# Autodesk Inventor assembly: Rama_siedziska
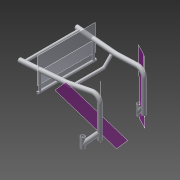
[picture p0: Inventor's stored thumbnail of the model, 180x180]
Saved by Autodesk Inventor 2015 (Build 190159000, 159)
## iProperties
Created: 2015-11-20
Part Number: Rama_siedziska
Document SubType Name: Konstrukcja spawana
Designer: graaapsik
Weld Material: Aluminium AW-7020
Author: graaapsik
## Documents named in this file (9)
- C:\Users\EriveltonDell\Documents\Centro Universitário da FEI\Wheelchair\CADEIRA DE RODAS - DESENHO\Model\Rama_siedziska.iam
- C:\Users\EriveltonDell\Documents\Centro Universitário da FEI\Wheelchair\CADEIRA DE RODAS - DESENHO\Model\Rura_podłużna_ergosiedziska_prawa.ipt
- C:\Users\EriveltonDell\Documents\Centro Universitário da FEI\Wheelchair\CADEIRA DE RODAS - DESENHO\Model\Rura_poprzeczna_ergosiedziska.ipt
- C:\Users\EriveltonDell\Documents\Centro Universitário da FEI\Wheelchair\CADEIRA DE RODAS - DESENHO\Model\Rura_poprzeczna_wygieta.ipt
- C:\Users\EriveltonDell\Documents\Centro Universitário da FEI\Wheelchair\CADEIRA DE RODAS - DESENHO\Model\Rura_podłużna_ergosiedziska_lewa.ipt
- C:\Users\EriveltonDell\Documents\Centro Universitário da FEI\Wheelchair\CADEIRA DE RODAS - DESENHO\Model\Rura_pionowa_kolka_przedniego.ipt
- C:\Users\EriveltonDell\Documents\Centro Universitário da FEI\Wheelchair\CADEIRA DE RODAS - DESENHO\Model\Rura_skosna_kolka_przedniego.ipt
- C:\Users\EriveltonDell\Documents\Centro Universitário da FEI\Wheelchair\CADEIRA DE RODAS - DESENHO\Model\Rura_pionowa_do_kol_tylnych.ipt
- C:\Users\EriveltonDell\Documents\Centro Universitário da FEI\Wheelchair\CADEIRA DE RODAS - DESENHO\Model\Belka.ipt
## Components (11 placed, 8 different names)
1. Rura_poprzeczna_ergosiedziska:1 — Równoległy:2, Równoległy:10, Zestawiający:1, Zestawiający:2, Zestawiający:3, Równoległy:11, Styczny:1, Zestawiający:4, Zestawiający:5, Zestawiający:7, Zestawiający:8, Zestawiający:29, Kąt:1
2. Rura_poprzeczna_wygieta:1 — Równoległy:10, Równoległy:12, Równoległy:13
3. Rura_podłużna_ergosiedziska_prawa:1 — Równoległy:2, Zestawiający:1, Zestawiający:2, Równoległy:13, Zestawiający:18, Zestawiający:22, Równoległy:14, Zestawiający:24, Zestawiający:25
4. Rura_podłużna_ergosiedziska_lewa:1 — Zestawiający:3, Równoległy:11, Styczny:1, Równoległy:12, Zestawiający:10, Zestawiający:16, Zestawiający:26, Zestawiający:27, Zestawiający:28, Równoległy:15
5. Rura_pionowa_kolka_przedniego:1 — Zestawiający:4, Zestawiający:5, Równoległy:16, Zestawiający:17, Zestawiający:23, Zestawiający:9
6. Rura_skosna_kolka_przedniego:1 — Zestawiający:21, Zestawiający:22, Zestawiający:23
7. Rura_pionowa_kolka_przedniego:2 — Zestawiający:7, Zestawiający:8, Zestawiający:9, Zestawiający:11, Zestawiający:15
8. Rura_skosna_kolka_przedniego:2 — Zestawiający:14, Zestawiający:15, Zestawiający:16
9. Rura_pionowa_do_kol_tylnych:1 — Równoległy:14, Zestawiający:24, Zestawiający:25, Symetria:1, Zestawiający:33
10. Rura_pionowa_do_kol_tylnych:2 — Zestawiający:26, Zestawiający:27, Zestawiający:28, Równoległy:15, Symetria:1, Zestawiający:32
11. Belka:1 — Zestawiający:29, Zestawiający:31, Równoległy:16
## Relationships (44: Mate 33, Flush 8, Tangent 1, Angle 1, Symmetry 1)
- Równoległy:2 [Flush]: Rura_poprzeczna_ergosiedziska:1 ↔ Rura_podłużna_ergosiedziska_prawa:1
- Równoległy:10 [Flush] (270 mm): Rura_poprzeczna_ergosiedziska:1 ↔ Rura_poprzeczna_wygieta:1
- Zestawiający:1 [Mate] (-30 mm): Rura_poprzeczna_ergosiedziska:1 ↔ Rura_podłużna_ergosiedziska_prawa:1
- Zestawiający:2 [Mate] (16 mm): Rura_poprzeczna_ergosiedziska:1 ↔ Rura_podłużna_ergosiedziska_prawa:1
- Zestawiający:3 [Mate] (-30 mm): Rura_poprzeczna_ergosiedziska:1 ↔ Rura_podłużna_ergosiedziska_lewa:1
- Równoległy:11 [Flush]: Rura_poprzeczna_ergosiedziska:1 ↔ Rura_podłużna_ergosiedziska_lewa:1
- Styczny:1 [Tangent]: Rura_poprzeczna_ergosiedziska:1 ↔ Rura_podłużna_ergosiedziska_lewa:1
- Równoległy:12 [Flush] (16 mm): Rura_poprzeczna_wygieta:1 ↔ Rura_podłużna_ergosiedziska_lewa:1
- Równoległy:13 [Flush] (16 mm): Rura_poprzeczna_wygieta:1 ↔ Rura_podłużna_ergosiedziska_prawa:1
- Zestawiający:4 [Mate] (450 mm): Rura_poprzeczna_ergosiedziska:1 ↔ Rura_pionowa_kolka_przedniego:1
- Zestawiający:5 [Mate] (-16 mm): Rura_poprzeczna_ergosiedziska:1 ↔ Rura_pionowa_kolka_przedniego:1
- Równoległy:16 [Flush] (-120 mm): Rura_pionowa_kolka_przedniego:1 ↔ Belka:1
- Zestawiający:7 [Mate] (416 mm): Rura_poprzeczna_ergosiedziska:1 ↔ Rura_pionowa_kolka_przedniego:2
- Zestawiający:8 [Mate] (450 mm): Rura_poprzeczna_ergosiedziska:1 ↔ Rura_pionowa_kolka_przedniego:2
- Zestawiający:9 [Mate]: Rura_pionowa_kolka_przedniego:1 ↔ Rura_pionowa_kolka_przedniego:2
- Zestawiający:10 [Mate]: Rura_podłużna_ergosiedziska_lewa:1
- Zestawiający:11 [Mate]: Rura_pionowa_kolka_przedniego:2
- Zestawiający:12 [Mate]
- Zestawiający:13 [Mate]
- Zestawiający:14 [Mate]: Rura_skosna_kolka_przedniego:2
- Zestawiający:15 [Mate] (16 mm): Rura_pionowa_kolka_przedniego:2 ↔ Rura_skosna_kolka_przedniego:2
- Zestawiający:16 [Mate] (16 mm): Rura_podłużna_ergosiedziska_lewa:1 ↔ Rura_skosna_kolka_przedniego:2
- Zestawiający:17 [Mate]: Rura_pionowa_kolka_przedniego:1
- Zestawiający:18 [Mate]: Rura_podłużna_ergosiedziska_prawa:1
- Zestawiający:19 [Mate]
- Zestawiający:20 [Mate]
- Zestawiający:21 [Mate]: Rura_skosna_kolka_przedniego:1
- Zestawiający:22 [Mate] (16 mm): Rura_podłużna_ergosiedziska_prawa:1 ↔ Rura_skosna_kolka_przedniego:1
- Zestawiający:23 [Mate] (16 mm): Rura_pionowa_kolka_przedniego:1 ↔ Rura_skosna_kolka_przedniego:1
- Równoległy:14 [Flush]: Rura_podłużna_ergosiedziska_prawa:1 ↔ Rura_pionowa_do_kol_tylnych:1
- Zestawiający:24 [Mate]: Rura_podłużna_ergosiedziska_prawa:1 ↔ Rura_pionowa_do_kol_tylnych:1
- Zestawiający:25 [Mate] (292.521 mm): Rura_podłużna_ergosiedziska_prawa:1 ↔ Rura_pionowa_do_kol_tylnych:1
- Zestawiający:26 [Mate]: Rura_podłużna_ergosiedziska_lewa:1 ↔ Rura_pionowa_do_kol_tylnych:2
- Zestawiający:27 [Mate] (292.521 mm): Rura_podłużna_ergosiedziska_lewa:1 ↔ Rura_pionowa_do_kol_tylnych:2
- Zestawiający:28 [Mate]: Rura_podłużna_ergosiedziska_lewa:1 ↔ Rura_pionowa_do_kol_tylnych:2
- Równoległy:15 [Flush]: Rura_podłużna_ergosiedziska_lewa:1 ↔ Rura_pionowa_do_kol_tylnych:2
- Zestawiający:29 [Mate] (-145 mm): Rura_poprzeczna_ergosiedziska:1 ↔ Belka:1
- Kąt:1 [Angle] (0 deg): Rura_poprzeczna_ergosiedziska:1
- Zestawiający:31 [Mate]: Belka:1
- Symetria:1 [Symmetry]: Rura_pionowa_do_kol_tylnych:1 ↔ Rura_pionowa_do_kol_tylnych:2
- Zestawiający:32 [Mate]: Rura_pionowa_do_kol_tylnych:2
- Zestawiający:33 [Mate]: Rura_pionowa_do_kol_tylnych:1
- Zestawiający:34 [Mate]
- Zestawiający:35 [Mate]
